# Autodesk Inventor assembly: RCR
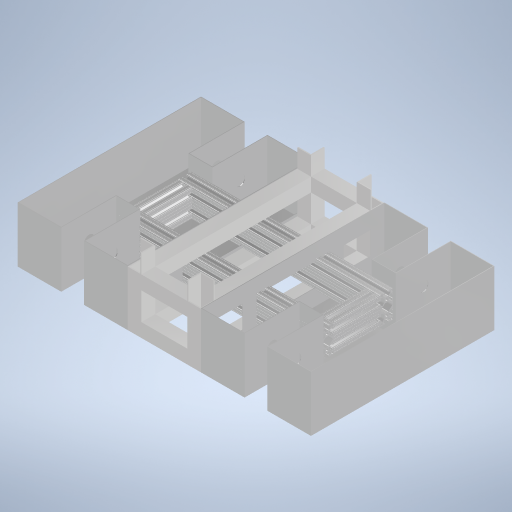
[picture p0: Inventor's stored thumbnail of the model, 512x512]
Saved by Autodesk Inventor 2023 (Build 270158000, 158)
## iProperties
Created: 2022-09-21
Part Number: RCR
Document SubType Name: Assembly
Designer: seene
Author: seene
## Documents named in this file (3)
- C:\Users\seene\Desktop\Stony Brook\SBRT\RoboRescue\Chassis\RCR.iam
- C:\Users\seene\Desktop\Stony Brook\SBRT\RoboRescue\Chassis\Frame\Chassis.iam
- C:\Users\seene\Desktop\Stony Brook\SBRT\RoboRescue\Chassis\DriveHousing\DriveHousing.ipt
## Components (3 placed, 2 different names)
1. Chassis:1 [sub-assembly] — Mate:1, Flush:1, Flush:2, Mate:2, Flush:3, Flush:4
2. DriveHousing:1 — Mate:1, Flush:1, Flush:2
3. DriveHousing:2 — Mate:2, Flush:3, Flush:4
## Relationships (6: Flush 4, Mate 2)
- Mate:1: Chassis:1 ↔ DriveHousing:1
- Flush:1: Chassis:1 ↔ DriveHousing:1
- Flush:2: Chassis:1 ↔ DriveHousing:1
- Mate:2: Chassis:1 ↔ DriveHousing:2
- Flush:3: Chassis:1 ↔ DriveHousing:2
- Flush:4: Chassis:1 ↔ DriveHousing:2
